# Autodesk Inventor assembly: frameortho
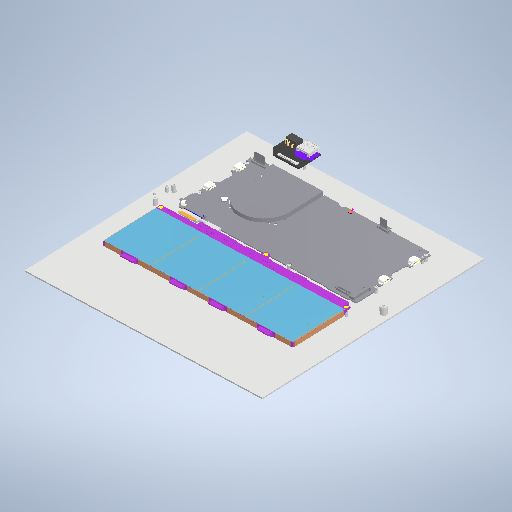
[picture p0: Inventor's stored thumbnail of the model, 512x512]
Saved by Autodesk Inventor 2025 (Build 290162010, 162A)
## iProperties
Created: 2026-01-15
Part Number: frameortho
Document SubType Name: Assembly
Designer: 200481997
Author: 200481997
## Documents named in this file (5)
- C:\Users\200481997\Documents\GitHub\frameergo\CAD\frameergo.iam
- C:\Users\200481997\Documents\GitHub\frameergo\CAD\Imports\Battery\FWKNAQ9_G01_20210911\Framework BatteryFWKNAQ9_G01_20210911.ipt
- C:\Users\200481997\Documents\GitHub\frameergo\CAD\chassis.ipt
- C:\Users\200481997\Documents\GitHub\frameergo\CAD\Imports\Motherboard\Framework Mobo\Framework Mobo.ipt
- C:\Users\200481997\Documents\GitHub\frameergo\CAD\Imports\DisplayPort Adapter\source\source.ipt
## Components (4 placed, 4 different names)
1. Framework Battery — Mate:5, Mate:6
2. Frameergo Chassis — Mate:1, Mate:2, Mate:3, Mate:4, Mate:5, Mate:6
3. Framework Mobo — Mate:1, Mate:2
4. DisplayPort Source Adapter — Mate:3, Mate:4
## Relationships (6: Mate 6)
- Mate:1: Frameergo Chassis ↔ Framework Mobo
- Mate:2: Frameergo Chassis ↔ Framework Mobo
- Mate:3: Frameergo Chassis ↔ DisplayPort Source Adapter
- Mate:4: Frameergo Chassis ↔ DisplayPort Source Adapter
- Mate:5: Framework Battery ↔ Frameergo Chassis
- Mate:6: Framework Battery ↔ Frameergo Chassis
